# Autodesk Inventor assembly: Ensamblajefinal
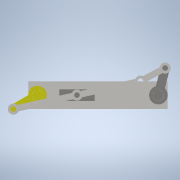
[picture p0: Inventor's stored thumbnail of the model, 180x180]
Saved by Autodesk Inventor 2020.5 (Build 245400000, 400)
## iProperties
Created: 2022-12-11
Part Number: Ensamblajefinal
Document SubType Name: Assembly
Designer: André Aguirre Apolo
Mass: 724.236 g
Surface Area: 393.727 cm^2
Volume: 92.1048 cm^3
Density: 7.86317 g/cm^3
Author: André Aguirre Apolo
## Documents named in this file (38)
- C:\Users\André Aguirre Apolo\Desktop\ESPOL\PAO2, 2022\Diseño y simulacion de maquinas\Teorico\proyecto\Ensamblajefinal.iam
- C:\Users\André Aguirre Apolo\Desktop\ESPOL\PAO2, 2022\Diseño y simulacion de maquinas\Teorico\proyecto\Bearing.ipt
- C:\Users\André Aguirre Apolo\Desktop\ESPOL\PAO2, 2022\Diseño y simulacion de maquinas\Teorico\proyecto\Crank2.ipt
- C:\Users\André Aguirre Apolo\Desktop\ESPOL\PAO2, 2022\Diseño y simulacion de maquinas\Teorico\proyecto\Conrod3.ipt
- C:\Users\André Aguirre Apolo\Desktop\ESPOL\PAO2, 2022\Diseño y simulacion de maquinas\Teorico\proyecto\Conrod2.ipt
- C:\Users\André Aguirre Apolo\Desktop\ESPOL\PAO2, 2022\Diseño y simulacion de maquinas\Teorico\proyecto\Crank1.ipt
- C:\Users\André Aguirre Apolo\Desktop\ESPOL\PAO2, 2022\Diseño y simulacion de maquinas\Teorico\proyecto\Runway.ipt
- C:\Users\André Aguirre Apolo\Desktop\ESPOL\PAO2, 2022\Diseño y simulacion de maquinas\Teorico\proyecto\Slider.ipt
- C:\Users\André Aguirre Apolo\Desktop\ESPOL\PAO2, 2022\Diseño y simulacion de maquinas\Teorico\proyecto\Ensamblajefinal\AIP\FEA\e6ifcojj4.fins
- C:\Users\André Aguirre Apolo\Desktop\ESPOL\PAO2, 2022\Diseño y simulacion de maquinas\Teorico\proyecto\Ensamblajefinal\AIP\FEA\e6ifcojj4.fsat
- C:\Users\André Aguirre Apolo\Desktop\ESPOL\PAO2, 2022\Diseño y simulacion de maquinas\Teorico\proyecto\Ensamblajefinal\AIP\FEA\e6ifcojj4.ftes
- C:\Users\André Aguirre Apolo\Desktop\ESPOL\PAO2, 2022\Diseño y simulacion de maquinas\Teorico\proyecto\Ensamblajefinal\AIP\FEA\e6ifcojj4.fwiz
- C:\Users\André Aguirre Apolo\Desktop\ESPOL\PAO2, 2022\Diseño y simulacion de maquinas\Teorico\proyecto\Ensamblajefinal\AIP\FEA\e6ifcojk0.fins
- C:\Users\André Aguirre Apolo\Desktop\ESPOL\PAO2, 2022\Diseño y simulacion de maquinas\Teorico\proyecto\Ensamblajefinal\AIP\FEA\e6ifcojk0.fsat
- C:\Users\André Aguirre Apolo\Desktop\ESPOL\PAO2, 2022\Diseño y simulacion de maquinas\Teorico\proyecto\Ensamblajefinal\AIP\FEA\e6ifcojk0.ftes
- C:\Users\André Aguirre Apolo\Desktop\ESPOL\PAO2, 2022\Diseño y simulacion de maquinas\Teorico\proyecto\Ensamblajefinal\AIP\FEA\e6ifcojk0.fwiz
- C:\Users\André Aguirre Apolo\Desktop\ESPOL\PAO2, 2022\Diseño y simulacion de maquinas\Teorico\proyecto\Ensamblajefinal\AIP\FEA\e6ifcojk1.fins
- C:\Users\André Aguirre Apolo\Desktop\ESPOL\PAO2, 2022\Diseño y simulacion de maquinas\Teorico\proyecto\Ensamblajefinal\AIP\FEA\e6ifcojk1.fsat
- C:\Users\André Aguirre Apolo\Desktop\ESPOL\PAO2, 2022\Diseño y simulacion de maquinas\Teorico\proyecto\Ensamblajefinal\AIP\FEA\e6ifcojk1.ftes
- C:\Users\André Aguirre Apolo\Desktop\ESPOL\PAO2, 2022\Diseño y simulacion de maquinas\Teorico\proyecto\Ensamblajefinal\AIP\FEA\e6ifcojk1.fwiz
- C:\Users\André Aguirre Apolo\Desktop\ESPOL\PAO2, 2022\Diseño y simulacion de maquinas\Teorico\proyecto\Ensamblajefinal\AIP\FEA\e6ifcojk2.fins
- C:\Users\André Aguirre Apolo\Desktop\ESPOL\PAO2, 2022\Diseño y simulacion de maquinas\Teorico\proyecto\Ensamblajefinal\AIP\FEA\e6ifcojk2.fsat
- C:\Users\André Aguirre Apolo\Desktop\ESPOL\PAO2, 2022\Diseño y simulacion de maquinas\Teorico\proyecto\Ensamblajefinal\AIP\FEA\e6ifcojk2.ftes
- C:\Users\André Aguirre Apolo\Desktop\ESPOL\PAO2, 2022\Diseño y simulacion de maquinas\Teorico\proyecto\Ensamblajefinal\AIP\FEA\e6ifcojkw.fwiz
- C:\Users\André Aguirre Apolo\Desktop\ESPOL\PAO2, 2022\Diseño y simulacion de maquinas\Teorico\proyecto\Ensamblajefinal\AIP\FEA\e6ifcojkx.fins
- C:\Users\André Aguirre Apolo\Desktop\ESPOL\PAO2, 2022\Diseño y simulacion de maquinas\Teorico\proyecto\Ensamblajefinal\AIP\FEA\e6ifcojkx.fsat
- C:\Users\André Aguirre Apolo\Desktop\ESPOL\PAO2, 2022\Diseño y simulacion de maquinas\Teorico\proyecto\Ensamblajefinal\AIP\FEA\e6ifcojkx.ftes
- C:\Users\André Aguirre Apolo\Desktop\ESPOL\PAO2, 2022\Diseño y simulacion de maquinas\Teorico\proyecto\Ensamblajefinal\AIP\FEA\e6ifcojkx.fwiz
- C:\Users\André Aguirre Apolo\Desktop\ESPOL\PAO2, 2022\Diseño y simulacion de maquinas\Teorico\proyecto\Ensamblajefinal\AIP\FEA\e6ifcojnk.fmsh
- C:\Users\André Aguirre Apolo\Desktop\ESPOL\PAO2, 2022\Diseño y simulacion de maquinas\Teorico\proyecto\Ensamblajefinal\AIP\FEA\e6ifcojnl.fres
- C:\Users\André Aguirre Apolo\Desktop\ESPOL\PAO2, 2022\Diseño y simulacion de maquinas\Teorico\proyecto\Ensamblajefinal\AIP\FEA\e6ifcojs0.fmsh
- C:\Users\André Aguirre Apolo\Desktop\ESPOL\PAO2, 2022\Diseño y simulacion de maquinas\Teorico\proyecto\Ensamblajefinal\AIP\FEA\e6ifcojs1.fres
- C:\Users\André Aguirre Apolo\Desktop\ESPOL\PAO2, 2022\Diseño y simulacion de maquinas\Teorico\proyecto\Ensamblajefinal\AIP\FEA\e6ifcojwg.fmsh
- C:\Users\André Aguirre Apolo\Desktop\ESPOL\PAO2, 2022\Diseño y simulacion de maquinas\Teorico\proyecto\Ensamblajefinal\AIP\FEA\e6ifcojwh.fres
- C:\Users\André Aguirre Apolo\Desktop\ESPOL\PAO2, 2022\Diseño y simulacion de maquinas\Teorico\proyecto\Ensamblajefinal\AIP\FEA\e6ifcok0w.fmsh
- C:\Users\André Aguirre Apolo\Desktop\ESPOL\PAO2, 2022\Diseño y simulacion de maquinas\Teorico\proyecto\Ensamblajefinal\AIP\FEA\e6ifcok0x.fres
- C:\Users\André Aguirre Apolo\Desktop\ESPOL\PAO2, 2022\Diseño y simulacion de maquinas\Teorico\proyecto\Ensamblajefinal\AIP\FEA\e6ifcok4g.fmsh
- C:\Users\André Aguirre Apolo\Desktop\ESPOL\PAO2, 2022\Diseño y simulacion de maquinas\Teorico\proyecto\Ensamblajefinal\AIP\FEA\e6ifcok5c.fres
## Components (8 placed, 7 different names)
1. Bearing:1 — Insertar:1, Nivelación:2, Coincidencia:1, Nivelación:3, Nivelación:4
2. Crank2:1 — Insertar:1, Insertar:2
3. Conrod3:1 — Insertar:2, Insertar:3, Insertar:6
4. Bearing:2 — Nivelación:2, Insertar:4, Coincidencia:2
5. Conrod2:1 — Insertar:3, Insertar:5
6. Crank1:1 — Insertar:4, Insertar:5
7. Runway:1 — Coincidencia:1, Nivelación:3, Coincidencia:2, Nivelación:4, Coincidencia:3
8. Slider:1 — Insertar:6, Coincidencia:3
## Relationships (12: Insert 6, Flush 3, Mate 3)
- Insertar:1: Bearing:1 ↔ Crank2:1
- Insertar:2: Crank2:1 ↔ Conrod3:1
- Nivelación:2 [Flush]: Bearing:1 ↔ Bearing:2
- Insertar:3: Conrod3:1 ↔ Conrod2:1
- Insertar:4: Bearing:2 ↔ Crank1:1
- Insertar:5: Conrod2:1 ↔ Crank1:1
- Coincidencia:1 [Mate]: Bearing:1 ↔ Runway:1
- Nivelación:3 [Flush]: Bearing:1 ↔ Runway:1
- Coincidencia:2 [Mate]: Bearing:2 ↔ Runway:1
- Insertar:6: Conrod3:1 ↔ Slider:1
- Nivelación:4 [Flush]: Bearing:1 ↔ Runway:1
- Coincidencia:3 [Mate]: Runway:1 ↔ Slider:1
## Named parameters: sa_8 = 279.477, sa_9 = 21.0779, sa_10 = 0, sa_11 = 0, sa_12 = 0, sa_13 = 9.51486, sa_14 = -131.6129 mm, sa_15 = 136.16094 mm, sa_16 = 113.81298 mm, sa_17 = 0, sa_18 = 0, sa_19 = -21.8797, sa_20 = -159.54181 mm, sa_21 = 125.20757 mm, sa_22 = 111.31298 mm, sa_23 = 7.20072, sa_24 = 1.24503, sa_25 = -17032, sa_29 = -131.6129 mm, sa_30 = 136.16094 mm, sa_31 = 116.31298 mm, sa_32 = 0.120084, sa_33 = -1.26289, sa_34 = 17032, sa_38 = -981, sa_39 = 0, sa_40 = 0, sa_41 = 0, sa_42 = 0 mm, sa_43 = 0 mm, sa_44 = 0 mm, sa_45 = 0, sa_46 = 7.36047, sa_47 = 115.102, sa_48 = 0, sa_49 = 0, sa_50 = 0, sa_51 = 4.60991, sa_52 = -182.91542 mm, sa_53 = 164.82201 mm, sa_54 = 113.81298 mm, sa_55 = 0, sa_56 = 0, sa_57 = 27.8975, sa_58 = -160.89162 mm, sa_59 = 185.19238 mm, sa_60 = 111.31298 mm, sa_61 = 8.6293, sa_62 = 3.08938, sa_63 = -17033.6, sa_67 = -182.91542 mm, sa_68 = 164.82201 mm, sa_69 = 116.31298 mm, sa_70 = -0.099391, sa_71 = -4.54903, sa_72 = 17033.6, sa_26 = -59.1812, sa_27 = -175.14, sa_28 = 0, sa_35 = 0, sa_36 = 0, sa_37 = 3.77282, sa_64 = -148.61023 mm, sa_65 = 117.54262 mm, sa_66 = 113.81298 mm, sa_73 = 0, sa_74 = 0, sa_75 = -37.1469, sa_76 = -177.2998 mm, sa_77 = 126.3124 mm, sa_78 = 111.31298 mm, sa_79 = 18.5453, sa_80 = -3.9962, sa_81 = -17045.3, sa_85 = -148.61023 mm, sa_86 = 117.54262 mm, sa_87 = 116.31298 mm, sa_88 = -9.44308, sa_89 = 5.00387, sa_90 = 17045.3, sa_102 = -78.716, sa_103 = 14.2207, sa_104 = 0, sa_105 = 0, sa_106 = 0, sa_107 = 7.50901, sa_108 = -175.29924 mm, sa_109 = 171.13943 mm, sa_110 = 113.81298 mm, sa_111 = 0, sa_112 = 0, sa_113 = 37.6463, sa_114 = -146.35919 mm, sa_115 = 179.04345 mm, sa_116 = 111.31298 mm, sa_117 = 13.9229, sa_118 = 2.00083, sa_119 = -17040.4, sa_123 = -175.29924 mm, sa_124 = 171.13943 mm, sa_125 = 116.31298 mm, sa_126 = -5.26788, sa_127 = -2.7938, sa_128 = 17040.4, sa_140 = -28.4167, sa_141 = 150.143, sa_142 = 0, sa_143 = 0, sa_144 = 0, sa_145 = 3.99652, sa_146 = -185.74564 mm, sa_147 = 160.9632 mm, sa_148 = 113.81298 mm, sa_149 = 0, sa_150 = 0, sa_151 = 11.7879, sa_152 = -166.49969 mm, sa_153 = 183.9761 mm, sa_154 = 111.31298 mm, sa_155 = 7.15442, sa_156 = 2.41509, sa_157 = -17031.6, sa_161 = -185.74564 mm, sa_162 = 160.9632 mm, sa_163 = 116.31298 mm, sa_164 = 1.62789, sa_165 = -3.98279, sa_166 = 17031.6
note: some values were not read from the file. Shown as the stored number, unit unknown: "sa_8", "sa_9", "sa_10", "sa_11", "sa_12", "sa_13", "sa_17", "sa_18", "sa_19", "sa_23", "sa_24", "sa_25", "sa_32", "sa_33", "sa_34", "sa_38", "sa_39", "sa_40", "sa_41", "sa_45", "sa_46", "sa_47", "sa_48", "sa_49", "sa_50", "sa_51", "sa_55", "sa_56", "sa_57", "sa_61", "sa_62", "sa_63", "sa_70", "sa_71", "sa_72", "sa_26", "sa_27", "sa_28", "sa_35", "sa_36", "sa_37", "sa_73", "sa_74", "sa_75", "sa_79", "sa_80", "sa_81", "sa_88", "sa_89", "sa_90", "sa_102", "sa_103", "sa_104", "sa_105", "sa_106", "sa_107", "sa_111", "sa_112", "sa_113", "sa_117", "sa_118", "sa_119", "sa_126", "sa_127", "sa_128", "sa_140", "sa_141", "sa_142", "sa_143", "sa_144", "sa_145", "sa_149", "sa_150", "sa_151", "sa_155", "sa_156", "sa_157", "sa_164", "sa_165", "sa_166".
